# Autodesk Inventor assembly: ASY MSC 2000 carriage
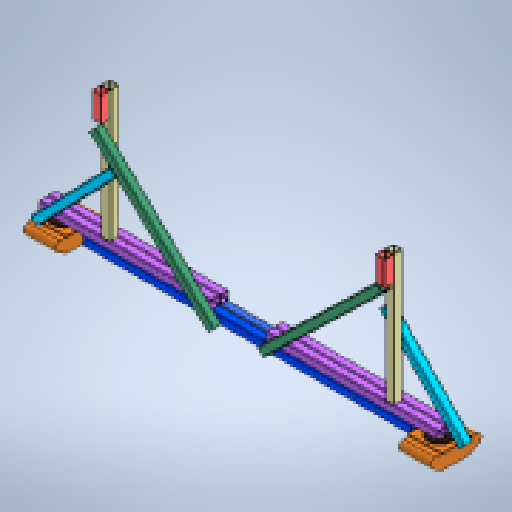
[picture p0: Inventor's stored thumbnail of the model, 512x512]
Saved by Autodesk Inventor 2025.1 (Build 291241020, 241B)
## iProperties
_SolveAssemblyDoc: Frame Generator Solve Assembly
_Version: 25.0.0
Created: 2024-11-20
Part Number: ASY MSC 2000 carriage
Document SubType Name: Assembly
Designer: user
Author: user
## Documents named in this file (4)
- C:\Users\user\YandexDisk-badmisterfox\домашниий пк\Inventor\Manturovo\Manturovo_Se-clar\ASY MSC 2000 carriage.iam
- C:\Users\user\YandexDisk-badmisterfox\домашниий пк\Inventor\Manturovo\Manturovo_Se-clar\MSC DIM 010 carriage.ipt
- C:\Users\user\YandexDisk-badmisterfox\домашниий пк\Inventor\Manturovo\Manturovo_Se-clar\ASY MSC 2000 carriage\Frame\Frame 1732110937978.iam
- C:\Users\user\YandexDisk-badmisterfox\домашниий пк\Inventor\Manturovo\Manturovo_Se-clar\3d party\roller platform.ipt
## Components (4 placed, 3 different names)
1. roller platform:2 — Mate:1, Mate:4, Flush:1
2. roller platform:1 — Mate:2, Mate:5
3. MSC DIM 010 carriage:1
4. Frame 1732110937978:1 [sub-assembly] — Mate:4, Flush:1, Mate:5
## Relationships (5: Mate 4, Flush 1)
- Mate:1: roller platform:2
- Mate:2: roller platform:1
- Mate:4: roller platform:2 ↔ Frame 1732110937978:1
- Flush:1: roller platform:2 ↔ Frame 1732110937978:1
- Mate:5: roller platform:1 ↔ Frame 1732110937978:1
